# Autodesk Inventor assembly: ZEndstop
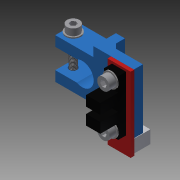
[picture p0: Inventor's stored thumbnail of the model, 180x180]
Saved by Autodesk Inventor 2015 SP1 (Build 190203100, 203)
## iProperties
Created: 2015-01-30
Part Number: ZEndstop
Document SubType Name: Assembly
Designer: Jack
Author: Jack
Title: Z Endstop
## Documents named in this file (6)
- C:\Users\Jack\ownCloud\Projects\CoreXY\InventorModel\ZAxis\ZEndstop.iam
- C:\Users\Jack\ownCloud\Projects\CoreXY\InventorModel\ZAxis\ZAxisEndstopMount.ipt
- C:\Users\Jack\ownCloud\Projects\CoreXY\InventorModel\Electronics\EndStops\EndStopOptical.ipt
- C:\Users\Jack\ownCloud\Projects\CoreXY\InventorModel\Hardware\BoltWashers\BoltWasher3\BoltWasher3x10.iam
- C:\Users\Jack\ownCloud\Projects\CoreXY\InventorModel\Hardware\Nuts\Nut3.ipt
- C:\Users\Jack\ownCloud\Projects\CoreXY\InventorModel\Hardware\BoltWashers\BoltWasher3\BoltWasher3x20.iam
## Components (8 placed, 5 different names)
1. ZAxisEndstopMount:1 — Mate:5, Mate:6, Mate:7, Angle:1, Angle:2, Mate:10, Mate:11, Mate:12, Mate:13, Angle:3, Mate:15
2. EndStopOptical:1 — Mate:1, Mate:2, Mate:3, Mate:4, Mate:7
3. BoltWasher3x10:1 [sub-assembly] — Mate:1, Mate:3, Mate:5, Mate:9
4. BoltWasher3x10:2 [sub-assembly] — Mate:2, Mate:4, Mate:6, Mate:8
5. Nut3:1 — Mate:8, Angle:2, Mate:11
6. Nut3:2 — Mate:9, Angle:1, Mate:10
7. Nut3:3 — Mate:14, Angle:3, Mate:15
8. BoltWasher3x20:1 [sub-assembly] — Mate:12, Mate:13, Mate:14
## Relationships (18: Mate 15, Angle 3)
- Mate:1: EndStopOptical:1 ↔ BoltWasher3x10:1
- Mate:2: EndStopOptical:1 ↔ BoltWasher3x10:2
- Mate:3: EndStopOptical:1 ↔ BoltWasher3x10:1
- Mate:4: EndStopOptical:1 ↔ BoltWasher3x10:2
- Mate:5: ZAxisEndstopMount:1 ↔ BoltWasher3x10:1
- Mate:6: ZAxisEndstopMount:1 ↔ BoltWasher3x10:2
- Mate:7: ZAxisEndstopMount:1 ↔ EndStopOptical:1
- Mate:8: BoltWasher3x10:2 ↔ Nut3:1
- Mate:9: BoltWasher3x10:1 ↔ Nut3:2
- Angle:1 (0 deg): ZAxisEndstopMount:1 ↔ Nut3:2
- Angle:2 (0 deg): ZAxisEndstopMount:1 ↔ Nut3:1
- Mate:10: ZAxisEndstopMount:1 ↔ Nut3:2
- Mate:11: ZAxisEndstopMount:1 ↔ Nut3:1
- Mate:12: ZAxisEndstopMount:1 ↔ BoltWasher3x20:1
- Mate:13: ZAxisEndstopMount:1 ↔ BoltWasher3x20:1
- Mate:14: Nut3:3 ↔ BoltWasher3x20:1
- Angle:3 (0 deg): ZAxisEndstopMount:1 ↔ Nut3:3
- Mate:15: ZAxisEndstopMount:1 ↔ Nut3:3
